# Autodesk Inventor assembly: MecanumFrame2
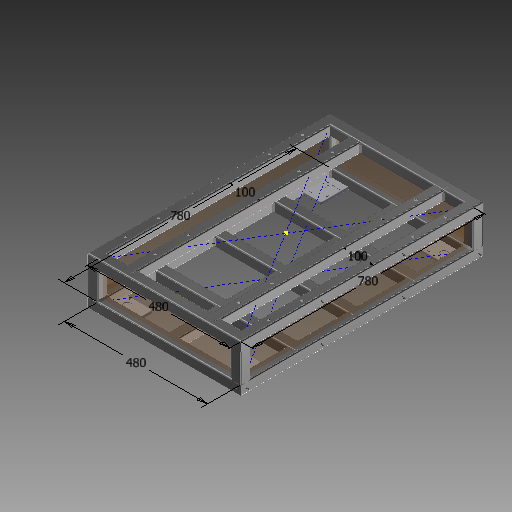
[picture p0: Inventor's stored thumbnail of the model, 512x512]
Saved by Autodesk Inventor 2018 (Build 220112000, 112)
## iProperties
Created: 2017-10-18
Part Number: MecanumFrame2
Document SubType Name: Weldment
Designer: Bryce Richards
Weld Material: Steel, Mild
Mass: 22429.4 g
Surface Area: 23297 cm^2
Volume: 2857.25 cm^3
Density: 7.85 g/cm^3
_SolveAssemblyDoc: Frame Generator Solve Assembly
_Version: 15.0.0
Author: Bryce Richards
## Documents named in this file (13)
- C:\Users\P136265\Documents\GitHub\mecanum-cad\MecanumFrame2.iam
- C:\Users\P136265\Documents\GitHub\mecanum-cad\MecanumWireframe2.ipt
- C:\Users\P136265\Documents\GitHub\mecanum-cad\MecanumFrame2\Frame\Frame0001.iam
- C:\Users\P136265\Documents\GitHub\mecanum-cad\Supports1.ipt
- C:\Users\P136265\Documents\GitHub\mecanum-cad\Crossmembers.ipt
- C:\Users\P136265\Documents\GitHub\mecanum-cad\CoverThread.ipt
- C:\Users\P136265\Documents\GitHub\mecanum-cad\bearing bracket for bolt screw.ipt
- C:\Users\P136265\Documents\GitHub\mecanum-cad\MecanumFrame2\AIP\FEA\caye7aykg.fins
- C:\Users\P136265\Documents\GitHub\mecanum-cad\MecanumFrame2\AIP\FEA\caye7aykg.fsat
- C:\Users\P136265\Documents\GitHub\mecanum-cad\MecanumFrame2\AIP\FEA\caye7aykg.ftes
- C:\Users\P136265\Documents\GitHub\mecanum-cad\MecanumFrame2\AIP\FEA\caye7aykg.fwiz
- C:\Users\P136265\Documents\GitHub\mecanum-cad\MecanumFrame2\AIP\FEA\caye7ayrk.fmsh
- C:\Users\P136265\Documents\GitHub\mecanum-cad\MecanumFrame2\AIP\FEA\caye7ayrl.fres
## Components (32 placed, 6 different names)
1. MecanumWireframe2:1
2. Frame0001:1 [sub-assembly] — Mate:1, Mate:2, Mate:3, Mate:4, Mate:5, Mate:6, Mate:7, Mate:8, Mate:9, Mate:10, Mate:11, Mate:12, Mate:13, Mate:14, Mate:15, Mate:16, Mate:17, Mate:18, Mate:19, Mate:20, Mate:21, Mate:22, Mate:23, Mate:24, Mate:25, Mate:26, Mate:27, Mate:28, Mate:29, Mate:30, Mate:31, Mate:32, Mate:33, Mate:34, Mate:35, Mate:36, Mate:37, Mate:38, Mate:39, Mate:40, Mate:41, Mate:42, Mate:43, Mate:44, Mate:45, Mate:46, Mate:47, Mate:48, Mate:49, Mate:50, Mate:51, Mate:52, Mate:53, Mate:54, Mate:55, Mate:56, Mate:57, Mate:58, Mate:59, Mate:60, Mate:61, Mate:62, Mate:63, Mate:64, Mate:65, Mate:66, Mate:67, Mate:68, Mate:69, Mate:70, Mate:71, Mate:72, Mate:73, Mate:74, Flush:3, Mate:75, Mate:76, Flush:4, Mate:77, Mate:78, Flush:5, Mate:79, Mate:80, Flush:6
3. Supports1:1 — Flush:1
4. Crossmembers:1 — Flush:2
5. CoverThread:1 — Mate:1, Mate:55, Mate:56
6. CoverThread:2 — Mate:2, Mate:59, Mate:60
7. CoverThread:3 — Mate:3, Mate:53, Mate:54
8. CoverThread:4 — Mate:4, Mate:57, Mate:58
9. CoverThread:5 — Mate:10, Mate:45, Mate:46
10. CoverThread:6 — Mate:8, Mate:49, Mate:50
11. CoverThread:7 — Mate:11, Mate:47, Mate:48
12. CoverThread:8 — Mate:9, Mate:51, Mate:52
13. CoverThread:9 — Mate:5, Mate:29, Mate:30
14. CoverThread:12 — Mate:6, Mate:31, Mate:32
15. CoverThread:13 — Mate:7, Mate:23, Mate:24
16. CoverThread:17 — Mate:12, Mate:37, Mate:38
17. CoverThread:20 — Mate:13, Mate:41, Mate:42
18. CoverThread:21 — Mate:14, Mate:43, Mate:44
19. CoverThread:22 — Mate:15, Mate:39, Mate:40
20. CoverThread:23 — Mate:16, Mate:35, Mate:36
21. CoverThread:24 — Mate:17, Mate:33, Mate:34
22. CoverThread:25 — Mate:18, Mate:27, Mate:28
23. CoverThread:26 — Mate:20, Mate:25, Mate:26
24. CoverThread:27 — Mate:19, Mate:21, Mate:22
25. CoverThread:28 — Mate:64, Mate:65, Mate:66
26. CoverThread:29 — Mate:61, Mate:62, Mate:63
27. CoverThread:30 — Mate:70, Mate:71, Mate:72
28. CoverThread:31 — Mate:67, Mate:68, Mate:69
29. bearing bracket for bolt screw:1 — Mate:73, Mate:74, Flush:3
30. bearing bracket for bolt screw:2 — Mate:75, Mate:76, Flush:4
31. bearing bracket for bolt screw:3 — Mate:79, Mate:80, Flush:6
32. bearing bracket for bolt screw:4 — Mate:77, Mate:78, Flush:5
## Relationships (86: Mate 80, Flush 6)
- Flush:1: Supports1:1
- Flush:2: Crossmembers:1
- Mate:1: Frame0001:1 ↔ CoverThread:1
- Mate:2: Frame0001:1 ↔ CoverThread:2
- Mate:3: Frame0001:1 ↔ CoverThread:3
- Mate:4: Frame0001:1 ↔ CoverThread:4
- Mate:5: Frame0001:1 ↔ CoverThread:9
- Mate:6: Frame0001:1 ↔ CoverThread:12
- Mate:7: Frame0001:1 ↔ CoverThread:13
- Mate:8: Frame0001:1 ↔ CoverThread:6
- Mate:9: Frame0001:1 ↔ CoverThread:8
- Mate:10: Frame0001:1 ↔ CoverThread:5
- Mate:11: Frame0001:1 ↔ CoverThread:7
- Mate:12: Frame0001:1 ↔ CoverThread:17
- Mate:13: Frame0001:1 ↔ CoverThread:20
- Mate:14: Frame0001:1 ↔ CoverThread:21
- Mate:15: Frame0001:1 ↔ CoverThread:22
- Mate:16: Frame0001:1 ↔ CoverThread:23
- Mate:17: Frame0001:1 ↔ CoverThread:24
- Mate:18: Frame0001:1 ↔ CoverThread:25
- Mate:19: Frame0001:1 ↔ CoverThread:27
- Mate:20: Frame0001:1 ↔ CoverThread:26
- Mate:21 (-270 mm): Frame0001:1 ↔ CoverThread:27
- Mate:22 (-17.5 mm): Frame0001:1 ↔ CoverThread:27
- Mate:23 (-17.5 mm): Frame0001:1 ↔ CoverThread:13
- Mate:24 (-17.5 mm): Frame0001:1 ↔ CoverThread:13
- Mate:25 (-17.5 mm): Frame0001:1 ↔ CoverThread:26
- Mate:26 (-17.5 mm): Frame0001:1 ↔ CoverThread:26
- Mate:27 (-270 mm): Frame0001:1 ↔ CoverThread:25
- Mate:28 (-17.5 mm): Frame0001:1 ↔ CoverThread:25
- Mate:29 (-17.5 mm): Frame0001:1 ↔ CoverThread:9
- Mate:30 (-17.5 mm): Frame0001:1 ↔ CoverThread:9
- Mate:31 (-17.5 mm): Frame0001:1 ↔ CoverThread:12
- Mate:32 (-17.5 mm): Frame0001:1 ↔ CoverThread:12
- Mate:33 (-270 mm): Frame0001:1 ↔ CoverThread:24
- Mate:34 (-17.5 mm): Frame0001:1 ↔ CoverThread:24
- Mate:35 (-270 mm): Frame0001:1 ↔ CoverThread:23
- Mate:36 (-17.5 mm): Frame0001:1 ↔ CoverThread:23
- Mate:37 (-17.5 mm): Frame0001:1 ↔ CoverThread:17
- Mate:38 (-17.5 mm): Frame0001:1 ↔ CoverThread:17
- Mate:39 (-17.5 mm): Frame0001:1 ↔ CoverThread:22
- Mate:40 (-17.5 mm): Frame0001:1 ↔ CoverThread:22
- Mate:41 (-17.5 mm): Frame0001:1 ↔ CoverThread:20
- Mate:42 (-17.5 mm): Frame0001:1 ↔ CoverThread:20
- Mate:43 (-17.5 mm): Frame0001:1 ↔ CoverThread:21
- Mate:44 (-17.5 mm): Frame0001:1 ↔ CoverThread:21
- Mate:45 (-17.5 mm): Frame0001:1 ↔ CoverThread:5
- Mate:46 (-17.5 mm): Frame0001:1 ↔ CoverThread:5
- Mate:47 (-17.5 mm): Frame0001:1 ↔ CoverThread:7
- Mate:48 (-17.5 mm): Frame0001:1 ↔ CoverThread:7
- Mate:49 (-17.5 mm): Frame0001:1 ↔ CoverThread:6
- Mate:50 (-17.5 mm): Frame0001:1 ↔ CoverThread:6
- Mate:51 (-17.5 mm): Frame0001:1 ↔ CoverThread:8
- Mate:52 (-17.5 mm): Frame0001:1 ↔ CoverThread:8
- Mate:53 (-17.5 mm): Frame0001:1 ↔ CoverThread:3
- Mate:54 (-17.5 mm): Frame0001:1 ↔ CoverThread:3
- Mate:55 (-17.5 mm): Frame0001:1 ↔ CoverThread:1
- Mate:56 (-17.5 mm): Frame0001:1 ↔ CoverThread:1
- Mate:57 (-17.5 mm): Frame0001:1 ↔ CoverThread:4
- Mate:58 (-17.5 mm): Frame0001:1 ↔ CoverThread:4
- Mate:59 (-17.5 mm): Frame0001:1 ↔ CoverThread:2
- Mate:60 (-17.5 mm): Frame0001:1 ↔ CoverThread:2
- Mate:61: Frame0001:1 ↔ CoverThread:29
- Mate:62 (-272 mm): Frame0001:1 ↔ CoverThread:29
- Mate:63 (-17.5 mm): Frame0001:1 ↔ CoverThread:29
- Mate:64: Frame0001:1 ↔ CoverThread:28
- Mate:65 (-17.5 mm): Frame0001:1 ↔ CoverThread:28
- Mate:66 (-272 mm): Frame0001:1 ↔ CoverThread:28
- Mate:67: Frame0001:1 ↔ CoverThread:31
- Mate:68 (-272 mm): Frame0001:1 ↔ CoverThread:31
- Mate:69 (-17.5 mm): Frame0001:1 ↔ CoverThread:31
- Mate:70: Frame0001:1 ↔ CoverThread:30
- Mate:71 (-272 mm): Frame0001:1 ↔ CoverThread:30
- Mate:72 (-17.5 mm): Frame0001:1 ↔ CoverThread:30
- Mate:73: Frame0001:1 ↔ bearing bracket for bolt screw:1
- Mate:74: Frame0001:1 ↔ bearing bracket for bolt screw:1
- Flush:3: Frame0001:1 ↔ bearing bracket for bolt screw:1
- Mate:75: Frame0001:1 ↔ bearing bracket for bolt screw:2
- Mate:76: Frame0001:1 ↔ bearing bracket for bolt screw:2
- Flush:4: Frame0001:1 ↔ bearing bracket for bolt screw:2
- Mate:77: Frame0001:1 ↔ bearing bracket for bolt screw:4
- Mate:78: Frame0001:1 ↔ bearing bracket for bolt screw:4
- Flush:5: Frame0001:1 ↔ bearing bracket for bolt screw:4
- Mate:79: Frame0001:1 ↔ bearing bracket for bolt screw:3
- Mate:80: Frame0001:1 ↔ bearing bracket for bolt screw:3
- Flush:6: Frame0001:1 ↔ bearing bracket for bolt screw:3
## Named parameters: sa_3 = 7.99e-11, sa_4 = -7.99e-11, sa_5 = 300000, sa_6 = 7.99e-11, sa_7 = 7.99e-11, sa_8 = 300000, sa_9 = -7.99e-11, sa_10 = -7.99e-11, sa_11 = 300000, sa_12 = -7.99e-11, sa_13 = 7.99e-11, sa_14 = 300000
note: some values were not read from the file. Shown as the stored number, unit unknown: "sa_3", "sa_4", "sa_5", "sa_6", "sa_7", "sa_8", "sa_9", "sa_10", "sa_11", "sa_12", "sa_13", "sa_14".
